# Autodesk Inventor assembly: 01001 ASY GBK wall shield Center 10
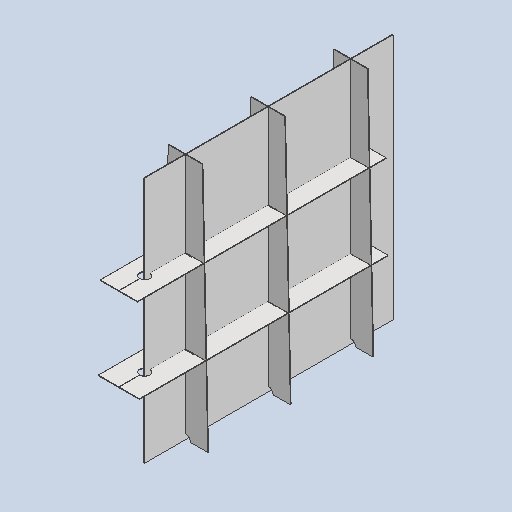
[picture p0: Inventor's stored thumbnail of the model, 512x512]
Saved by Autodesk Inventor 2026.2 (Build 302298000, 298)
## iProperties
Created: 2026-05-19
Part Number: 01001 ASY GBK wall shield Center 10
Document SubType Name: Assembly
Designer: pokla
Mass: 123029 g
Surface Area: 79995.2 cm^2
Volume: 15672.5 cm^3
Density: 7.85 g/cm^3
Author: admin
## Documents named in this file (5)
- C:\Users\pokla\Documents\Inventor\GBK-Gubkinskiy\01001 ASY GBK wall shield Center 10.iam
- C:\Users\pokla\Documents\Inventor\GBK-Gubkinskiy\01011 GBK Center rib 3.ipt
- C:\Users\pokla\Documents\Inventor\GBK-Gubkinskiy\01013 GBK stringer C7.ipt
- C:\Users\pokla\Documents\Inventor\GBK-Gubkinskiy\010.7 GBK shield.ipt
- C:\Users\pokla\Documents\Inventor\GBK-Gubkinskiy\01014 GBK stringer C8.ipt
## Components (11 placed, 4 different names)
1. 01013 GBK stringer C7:1 — Rigid:1
2. 010.7 GBK shield:1 — Mate:1, Flush:1, Mate:2, Mate:5, Flush:5, Mate:4, Flush:6, Flush:7
3. 01014 GBK stringer C8:1 — Rigid:2
4. 01013 GBK stringer C7:2 — Rigid:4
5. 01014 GBK stringer C8:2 — Rigid:3
6. 01011 GBK Center rib 3:2 — Mate:4, Flush:4, Flush:6, Rigid:3, Rigid:4
7. 01011 GBK Center rib 3:1 — Mate:5, Flush:5, Flush:4, Flush:7, Rigid:1, Rigid:2
8. 01011 GBK Center rib 3:3
9. 01011 GBK Center rib 3:4
10. 01011 GBK Center rib 3:5
11. 01011 GBK Center rib 3:6
## Component patterns: (3 elements, first: 01011 GBK Center rib 3:2 + 01011 GBK Center rib 3:1)
## Relationships (13: Flush 5, Mate 4, WeldJoint 4)
- Mate:1: 010.7 GBK shield:1
- Flush:1: 010.7 GBK shield:1
- Mate:2: 010.7 GBK shield:1
- Mate:5: 010.7 GBK shield:1 ↔ 01011 GBK Center rib 3:1
- Flush:5 (250 mm): 010.7 GBK shield:1 ↔ 01011 GBK Center rib 3:1
- Mate:4: 010.7 GBK shield:1 ↔ 01011 GBK Center rib 3:2
- Flush:4: 01011 GBK Center rib 3:2 ↔ 01011 GBK Center rib 3:1
- Flush:6: 010.7 GBK shield:1 ↔ 01011 GBK Center rib 3:2
- Flush:7: 010.7 GBK shield:1 ↔ 01011 GBK Center rib 3:1
- Rigid:1 [WeldJoint] (4 mm): 01013 GBK stringer C7:1 ↔ 01011 GBK Center rib 3:1
- Rigid:2 [WeldJoint] (4 mm): 01014 GBK stringer C8:1 ↔ 01011 GBK Center rib 3:1
- Rigid:3 [WeldJoint]: 01014 GBK stringer C8:2 ↔ 01011 GBK Center rib 3:2
- Rigid:4 [WeldJoint]: 01013 GBK stringer C7:2 ↔ 01011 GBK Center rib 3:2
